# Autodesk Inventor assembly: carrier
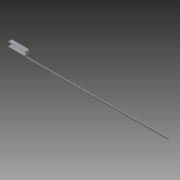
[picture p0: Inventor's stored thumbnail of the model, 180x180]
Saved by Autodesk Inventor 2013 (Build 170138000, 138)
## iProperties
Created: 2013-01-17
Part Number: carrier
Document SubType Name: Assembly
Designer: istvan.burbank
Author: istvan.burbank
## Documents named in this file (4)
- C:\Users\istvan.burbank\Documents\GitHub\Crown-Fire\CAD\Electronics\carrier\carrier.iam
- C:\Users\istvan.burbank\Documents\GitHub\Crown-Fire\CAD\Electronics\carrier\carrier20.iam
- C:\Users\istvan.burbank\Documents\GitHub\Crown-Fire\CAD\Electronics\carrier\carrier12.iam
- C:\Users\istvan.burbank\Documents\GitHub\Crown-Fire\CAD\Electronics\carrier\guide.ipt
## Components (6 placed, 3 different names)
1. carrier20:1 [sub-assembly] — Mate:1, Mate:2, Mate:9, Flush:1
2. carrier20:2 [sub-assembly] — Mate:1, Mate:2, Mate:3, Mate:4
3. carrier20:3 [sub-assembly] — Mate:3, Mate:4, Mate:5, Mate:6
4. carrier20:4 [sub-assembly] — Mate:5, Mate:6, Mate:7, Mate:8
5. carrier12:1 [sub-assembly] — Mate:7, Mate:8
6. guide:1 — Mate:9, Flush:1
## Relationships (10: Mate 9, Flush 1)
- Mate:1: carrier20:1 ↔ carrier20:2
- Mate:2: carrier20:1 ↔ carrier20:2
- Mate:3: carrier20:2 ↔ carrier20:3
- Mate:4: carrier20:2 ↔ carrier20:3
- Mate:5: carrier20:3 ↔ carrier20:4
- Mate:6: carrier20:3 ↔ carrier20:4
- Mate:7: carrier20:4 ↔ carrier12:1
- Mate:8: carrier20:4 ↔ carrier12:1
- Mate:9: carrier20:1 ↔ guide:1
- Flush:1: carrier20:1 ↔ guide:1
